# Autodesk Inventor assembly: Control_Panel
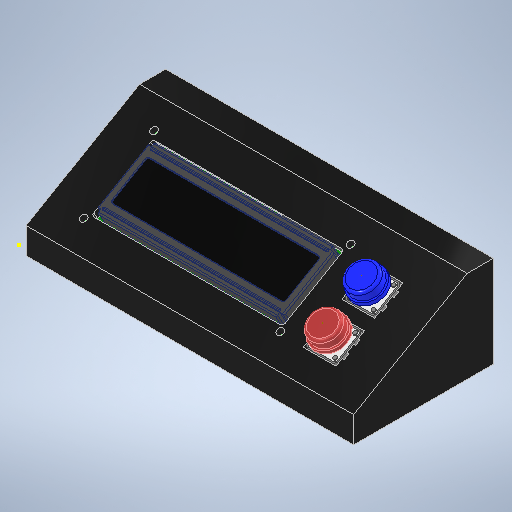
[picture p0: Inventor's stored thumbnail of the model, 512x512]
Saved by Autodesk Inventor 2025.1 (Build 291241020, 241B)
## iProperties
Created: 2024-11-21
Part Number: Control_Panel
Document SubType Name: Assembly
Designer: leon-
Author: leon-
## Documents named in this file (5)
- C:\Users\leon-\OneDrive\Dokumente\Education\Berkeley\Embedded_Systems\Project\MagDrop4\CAD_Model\Control_Panel.iam
- C:\Users\leon-\OneDrive\Dokumente\Education\Berkeley\Embedded_Systems\Project\MagDrop4\CAD_Model\Purchase_Parts\Electronics\Display.ipt
- C:\Users\leon-\OneDrive\Dokumente\Education\Berkeley\Embedded_Systems\Project\MagDrop4\CAD_Model\3DPrint_Parts\Control_Mount.ipt
- C:\Users\leon-\OneDrive\Dokumente\Education\Berkeley\Embedded_Systems\Project\MagDrop4\CAD_Model\3DPrint_Parts\M2-5_Nut.ipt
- C:\Users\leon-\OneDrive\Dokumente\Education\Berkeley\Embedded_Systems\Project\MagDrop4\CAD_Model\Purchase_Parts\Electronics\Tactile_Button\Tactile_Button.iam
## Components (8 placed, 4 different names)
1. Display:1 — Mate:1, Mate:2, Mate:3, Mate:5, Mate:6, Mate:7, Mate:8
2. Control_Mount:1 — Mate:1, Mate:2, Mate:3, Mate:4, Mate:9, Mate:10, Mate:11, Mate:12, Mate:13, Mate:14
3. M2-5_Nut:1 — Mate:4, Mate:8, Flush:1
4. M2-5_Nut:2 — Mate:5, Flush:2
5. M2-5_Nut:3 — Mate:6, Flush:3
6. M2-5_Nut:4 — Mate:7, Flush:1, Flush:2, Flush:3
7. Tactile_Button:1 [sub-assembly] — Mate:9, Mate:10, Mate:11
8. Tactile_Button:2 [sub-assembly] — Mate:12, Mate:13, Mate:14
## Relationships (17: Mate 14, Flush 3)
- Mate:1: Display:1 ↔ Control_Mount:1
- Mate:2: Display:1 ↔ Control_Mount:1
- Mate:3: Display:1 ↔ Control_Mount:1
- Mate:4: Control_Mount:1 ↔ M2-5_Nut:1
- Mate:5: Display:1 ↔ M2-5_Nut:2
- Mate:6: Display:1 ↔ M2-5_Nut:3
- Mate:7: Display:1 ↔ M2-5_Nut:4
- Mate:8: Display:1 ↔ M2-5_Nut:1
- Flush:1: M2-5_Nut:1 ↔ M2-5_Nut:4
- Flush:2: M2-5_Nut:2 ↔ M2-5_Nut:4
- Flush:3: M2-5_Nut:3 ↔ M2-5_Nut:4
- Mate:9: Control_Mount:1 ↔ Tactile_Button:1
- Mate:10 (0.25 mm): Control_Mount:1 ↔ Tactile_Button:1
- Mate:11 (0.25 mm): Control_Mount:1 ↔ Tactile_Button:1
- Mate:12: Control_Mount:1 ↔ Tactile_Button:2
- Mate:13 (0.25 mm): Control_Mount:1 ↔ Tactile_Button:2
- Mate:14 (0.25 mm): Control_Mount:1 ↔ Tactile_Button:2
